# Autodesk Inventor assembly: SpurFixed
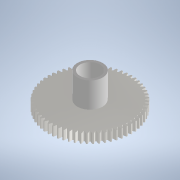
[picture p0: Inventor's stored thumbnail of the model, 180x180]
Saved by Autodesk Inventor 2022 (Build 260153000, 153)
## iProperties
Created: 2023-02-07
Part Number: SpurFixed
Document SubType Name: Assembly
Designer: Deven Joshi
Author: Deven Joshi
## Documents named in this file (3)
- C:\Users\ac_jo\OneDrive\Documents\TA202\SpurFixed.iam
- C:\Users\ac_jo\OneDrive\Documents\TA202\SpurFixed\Design Accelerator\Spur Gears1.iam
- C:\Users\ac_jo\OneDrive\Documents\TA202\collar.ipt
## Components (2 placed, 2 different names)
1. Spur Gears:1 [sub-assembly] — Mate:1, Mate:2
2. collar:1 — Mate:1, Mate:2
## Relationships (2: Mate 2)
- Mate:1: Spur Gears:1 ↔ collar:1
- Mate:2: Spur Gears:1 ↔ collar:1
